# Autodesk Inventor assembly: tsop
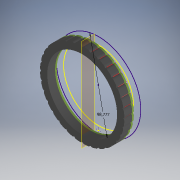
[picture p0: Inventor's stored thumbnail of the model, 180x180]
Saved by Autodesk Inventor 2020 (Build 240168000, 168)
## iProperties
Created: 2024-11-04
Part Number: tsop
Document SubType Name: Assembly
Designer: Ivan
Mass: 61.2553 g
Surface Area: 302.446 cm^2
Volume: 25.5389 cm^3
Density: 2.39851 g/cm^3
Author: Ivan
## Documents named in this file (4)
- C:\!projects\DASH-\3D\Dash-V1\tsop.iam
- C:\!projects\DASH-\3D\Dash-V1\tsop_lid.ipt
- C:\!projects\DASH-\3D\Dash-V1\step\tssp58038.ipt
- C:\!projects\DASH-\3D\Dash-V1\tsop_board.ipt
## Components (34 placed, 3 different names)
1. tsop_lid:1 — Совмещение:1, Заподлицо:1, Угол:1, Угол:2, Угол:3, Совмещение:2, Совмещение:3, Совмещение:4, Вставка:1, Вставка:2
2. tsop_board:1 — Вставка:1, Вставка:2
3. tssp58038:1 — Угол:1, Угол:3, Совмещение:2, Совмещение:3, Совмещение:4
4. tssp58038:2
5. tssp58038:3
6. tssp58038:4
7. tssp58038:5
8. tssp58038:6
9. tssp58038:7
10. tssp58038:8
11. tssp58038:9
12. tssp58038:10
13. tssp58038:11
14. tssp58038:12
15. tssp58038:13
16. tssp58038:14
17. tssp58038:15
18. tssp58038:16
19. tssp58038:17
20. tssp58038:18
21. tssp58038:19
22. tssp58038:20
23. tssp58038:21
24. tssp58038:22
25. tssp58038:23
26. tssp58038:24
27. tssp58038:25
28. tssp58038:26
29. tssp58038:27
30. tssp58038:28
31. tssp58038:29
32. tssp58038:30
33. tssp58038:31
34. tssp58038:32
## Component patterns: (32 elements, first: tssp58038:1)
## Relationships (10: Mate 4, Angle 3, Insert 2, Flush 1)
- Совмещение:1 [Mate]: tsop_lid:1
- Заподлицо:1 [Flush]: tsop_lid:1
- Угол:1 [Angle] (0 deg): tsop_lid:1 ↔ tssp58038:1
- Угол:2 [Angle] (0 deg): tsop_lid:1
- Угол:3 [Angle] (0 deg): tsop_lid:1 ↔ tssp58038:1
- Совмещение:2 [Mate]: tsop_lid:1 ↔ tssp58038:1
- Совмещение:3 [Mate]: tsop_lid:1 ↔ tssp58038:1
- Совмещение:4 [Mate]: tsop_lid:1 ↔ tssp58038:1
- Вставка:1 [Insert]: tsop_lid:1 ↔ tsop_board:1
- Вставка:2 [Insert]: tsop_lid:1 ↔ tsop_board:1
